# Autodesk Inventor assembly: 578162 VUVG-L10-M52-MT-M5-1H2L-W1
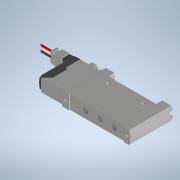
[picture p0: Inventor's stored thumbnail of the model, 180x180]
Saved by Autodesk Inventor 2021 (Build 250183000, 183)
## iProperties
Category: PARTsolutions
Company: FESTO
Created: 2026-04-25
Part Number: 578162 VUVG-L10-M52-MT-M5-1H2L-W1
Catalog Web Link: www.3dfindit.com
Description: VUVG-solenoid valve
Vendor: FESTO
Document SubType Name: Assembly
Designer: psAdmin
Manufacturer: FESTO
Mass: 44 g
Surface Area: 97.2554 cm^2
Volume: 19.4952 cm^3
Density: 2.25697 g/cm^3
Title: 578162 VUVG-L10-M52-MT-M5-1H2L-W1
Author: Cadenas PARTsolutions
Comments: solenoid valve
PSOL_IDENT_0: {ATYP=ASSISTANT},{DATA=script=$CADENAS_DATA/23d-libs/festo/webfesto.vbb&M_FAMILY=VUVG&M_GROUP=01&M_P
PSOL_IDENT_1: ARTNO=578162&IDCODE1=VUVG-L10-M52-MT-M5-1H2L-W1&IDCODE2=&customer_number_cns=&MATES=1&LOD=HI&LOCKERP=
PSOL_IDENT_2: 0&SINGLEPART=1}
NB: 578162 VUVG-L10-M52-MT-M5-1H2L-W1
NN: VUVG
NT: solenoid valve
NBSYN: $TNR. $TYP.
LINA: 578162 VUVG-L10-M52-MT-M5-1H2L-W1
CATALOG: Festo
TNR: 578162
TYP: VUVG-L10-M52-MT-M5-1H2L-W1
CNSMASSEXACT: 0.044
GTIN: 4052568104801
REACH: Yes
REACHSVHC: No
REACHHAZSUBS: -
REACHSCIP: -
REACHVALDATE: -
SUPPLIER: FESTO
ARTICLENO: 578162 VUVG-L10-M52-MT-M5-1H2L-W1
BOMINFO: 578162 VUVG-L10-M52-MT-M5-1H2L-W1
CREATOR: CADENAS GmbH
## Documents named in this file (4)
- e:\temp\worker_COMMON_215\temp\tmp_4624_0_IhsmB\format_0\578162 VUVG-L10-M52-MT-M5-1H2L-W1.iam
- e:\temp\worker_COMMON_215\temp\tmp_4624_0_IhsmB\format_0\564212 VUVG-L-10-M52-M-T-M5--1H2--L-W1---(G).ipt
- e:\temp\worker_COMMON_215\temp\tmp_4624_0_IhsmB\format_0\566714 VAVE-L1-1VH2-LP.ipt
- e:\temp\worker_COMMON_215\temp\tmp_4624_0_IhsmB\format_0\566654 NEBV-H1G2-KN-0_5-N-LE2.ipt
## Components (3 placed, 3 different names)
1. 564212 VUVG-L-10-M52-M-T-M5--1H2--L-W1---(G):1 — VAVE1_XY@1 <-> VAVE_XY@2, VAVE1_Z@1 <-> VAVE_Z@2, VAVE1_YZ@1 <-> VAVE_YZ@2
2. 566714 VAVE-L1-1VH2-LP:1 — VAVE1_XY@1 <-> VAVE_XY@2, VAVE1_Z@1 <-> VAVE_Z@2, VAVE1_YZ@1 <-> VAVE_YZ@2, NEBV_XY@2 <-> NEBV_XY@3, NEBV_Z@2 <-> NEBV_Z@3, NEBV_YZ@2 <-> NEBV_YZ@3
3. 566654 NEBV-H1G2-KN-0_5-N-LE2:1 — NEBV_XY@2 <-> NEBV_XY@3, NEBV_Z@2 <-> NEBV_Z@3, NEBV_YZ@2 <-> NEBV_YZ@3
## Relationships (6: Mate 4, Angle 2)
- VAVE1_XY@1 <-> VAVE_XY@2 [Mate]: 564212 VUVG-L-10-M52-M-T-M5--1H2--L-W1---(G):1 ↔ 566714 VAVE-L1-1VH2-LP:1
- VAVE1_Z@1 <-> VAVE_Z@2 [Mate]: 564212 VUVG-L-10-M52-M-T-M5--1H2--L-W1---(G):1 ↔ 566714 VAVE-L1-1VH2-LP:1
- VAVE1_YZ@1 <-> VAVE_YZ@2 [Angle] (180 deg): 564212 VUVG-L-10-M52-M-T-M5--1H2--L-W1---(G):1 ↔ 566714 VAVE-L1-1VH2-LP:1
- NEBV_XY@2 <-> NEBV_XY@3 [Mate]: 566714 VAVE-L1-1VH2-LP:1 ↔ 566654 NEBV-H1G2-KN-0_5-N-LE2:1
- NEBV_Z@2 <-> NEBV_Z@3 [Mate]: 566714 VAVE-L1-1VH2-LP:1 ↔ 566654 NEBV-H1G2-KN-0_5-N-LE2:1
- NEBV_YZ@2 <-> NEBV_YZ@3 [Angle] (0 deg): 566714 VAVE-L1-1VH2-LP:1 ↔ 566654 NEBV-H1G2-KN-0_5-N-LE2:1
